# Autodesk Inventor assembly: ArmsAssembly
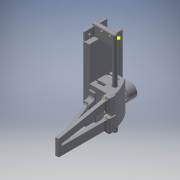
[picture p0: Inventor's stored thumbnail of the model, 180x180]
Saved by Autodesk Inventor 2018 (Build 220112000, 112)
## iProperties
Created: 2018-10-19
Part Number: ArmsAssembly
Document SubType Name: Assembly
Designer: reide
Author: reide
## Documents named in this file (9)
- C:\Users\reide\OneDrive\Documents\Inventor\TSA\2019\Animatronics\Glyptodon\Glyptodon Work\ArmsAssembly.iam
- C:\Users\reide\OneDrive\Documents\Inventor\TSA\2019\Animatronics\Glyptodon\Turtle Work\arms\Supporter.ipt
- C:\Users\reide\OneDrive\Documents\Inventor\TSA\2019\Animatronics\Glyptodon\Mock Parts\servo (2)_MIR.ipt
- C:\Users\reide\OneDrive\Documents\Inventor\TSA\2019\Animatronics\Glyptodon\Glyptodon Work\Arms\Rack.ipt
- C:\Users\reide\OneDrive\Documents\Inventor\TSA\2019\Animatronics\Glyptodon\Glyptodon Work\Arms\Roller_Wheel.ipt
- C:\Users\reide\OneDrive\Documents\Inventor\TSA\2019\Animatronics\Glyptodon\Glyptodon Work\Arms\ArmTruss.iam
- C:\Users\reide\OneDrive\Documents\Inventor\TSA\2019\Animatronics\Glyptodon\Glyptodon Work\Arms\ArmRod.ipt
- C:\Users\reide\OneDrive\Documents\Inventor\TSA\2019\Animatronics\Glyptodon\Glyptodon Work\Arms\GuideArmConnector.ipt
- C:\Users\reide\OneDrive\Documents\Inventor\TSA\2019\Animatronics\Glyptodon\Glyptodon Work\Arms\GuideArmConnectorLimitSwitch.ipt
## Components (8 placed, 8 different names)
1. Supporter:1 — Flush:12, Mate:20, Flush:14, Flush:16, Flush:17, Mate:23, Flush:18, Mate:24, Flush:19, Flush:20
2. servo (2)_MIR:1 — Mate:17, Mate:18, Mate:19, Mate:21, Flush:15, Mate:26
3. Rack:1 — Flush:12, Mate:17, Flush:20
4. Roller_Wheel:2 — Mate:18, Mate:19
5. ArmTruss:1 [sub-assembly] — Mate:20, Flush:14, Mate:21, Flush:15, Mate:22, Mate:26
6. ArmRod:1 — Mate:22, Mate:25
7. GuideArmConnector:1 — Flush:16, Flush:17, Mate:23, Mate:25
8. GuideArmConnectorLimitSwitch:1 — Flush:18, Mate:24, Flush:19
## Relationships (18: Mate 10, Flush 8)
- Flush:12: Supporter:1 ↔ Rack:1
- Mate:17: servo (2)_MIR:1 ↔ Rack:1
- Mate:18: servo (2)_MIR:1 ↔ Roller_Wheel:2
- Mate:19: servo (2)_MIR:1 ↔ Roller_Wheel:2
- Mate:20: Supporter:1 ↔ ArmTruss:1
- Flush:14: Supporter:1 ↔ ArmTruss:1
- Mate:21 (0.5 mm): servo (2)_MIR:1 ↔ ArmTruss:1
- Flush:15: servo (2)_MIR:1 ↔ ArmTruss:1
- Mate:22: ArmTruss:1 ↔ ArmRod:1
- Flush:16: Supporter:1 ↔ GuideArmConnector:1
- Flush:17: Supporter:1 ↔ GuideArmConnector:1
- Mate:23: Supporter:1 ↔ GuideArmConnector:1
- Flush:18: Supporter:1 ↔ GuideArmConnectorLimitSwitch:1
- Mate:24: Supporter:1 ↔ GuideArmConnectorLimitSwitch:1
- Flush:19: Supporter:1 ↔ GuideArmConnectorLimitSwitch:1
- Mate:25: ArmRod:1 ↔ GuideArmConnector:1
- Mate:26: servo (2)_MIR:1 ↔ ArmTruss:1
- Flush:20 (6.361 mm): Supporter:1 ↔ Rack:1
